# Autodesk Inventor assembly: G40
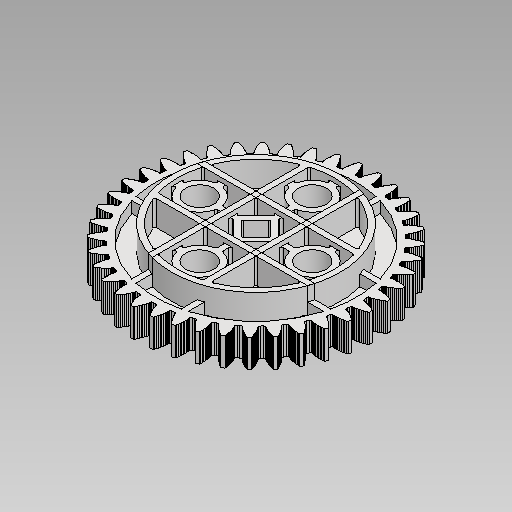
[picture p0: Inventor's stored thumbnail of the model, 512x512]
Saved by Autodesk Inventor 2020 (Build 240168000, 168)
## iProperties
Created: 2019-05-06
Part Number: G40
Document SubType Name: Assembly
Designer: Varga Daniel
Author: Varga Daniel
## Documents named in this file (3)
- C:\!_Dani\!_cloud\OneDrive\!_munka\Revolution\StructuralParts\Gears\G40.iam
- C:\!_Dani\!_cloud\OneDrive\!_munka\Revolution\StructuralParts\Gears\gear40_tooth.ipt
- C:\!_Dani\!_cloud\OneDrive\!_munka\Revolution\StructuralParts\Gears\Gear central part.iam
## Components (2 placed, 2 different names)
1. gear40_tooth:1 — Mate:1, Flush:1, Mate:2
2. Gear central part:1 [sub-assembly] — Mate:1, Flush:1, Mate:2
## Relationships (3: Mate 2, Flush 1)
- Mate:1: gear40_tooth:1 ↔ Gear central part:1
- Flush:1: gear40_tooth:1 ↔ Gear central part:1
- Mate:2: gear40_tooth:1 ↔ Gear central part:1
